# Autodesk Inventor assembly: GateLessMaterialAssembly
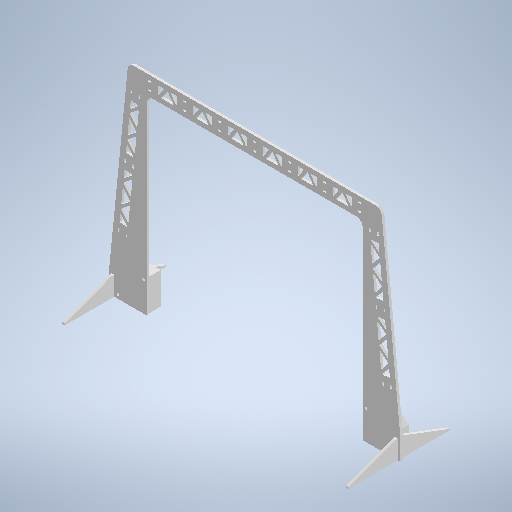
[picture p0: Inventor's stored thumbnail of the model, 512x512]
Saved by Autodesk Inventor 2025.1 (Build 291241000, 241)
## iProperties
Created: 2025-03-30
Part Number: GateLessMaterialAssembly
Document SubType Name: Assembly
Designer: 42060
Author: 42060
## Documents named in this file (4)
- C:\Users\42060\Desktop\School\Projects\RoboClash\LineFollower_Gate\GateLessMaterial\GateLessMaterialAssembly.iam
- C:\Users\42060\Desktop\School\Projects\RoboClash\LineFollower_Gate\GateLessMaterial\GateBrigeSideLessMaterial.ipt
- C:\Users\42060\Desktop\School\Projects\RoboClash\LineFollower_Gate\GateLessMaterial\LegLessMaterial.ipt
- C:\Users\42060\Desktop\School\Projects\RoboClash\LineFollower_Gate\GateLessMaterial\Sensor.ipt
## Components (5 placed, 3 different names)
1. GateBrigeSideLessMaterial:1 — Vložit:1, Vložit:2, Vložit:3, Vložit:4, Proti sobě:1, Proti sobě:2, Proti sobě:3, Proti sobě:4, Proti sobě:5, Proti sobě:6
2. LegLessMaterial:1 — Proti sobě:1, Proti sobě:2, Proti sobě:3
3. Sensor:1 — Vložit:1, Vložit:2
4. Sensor:2 — Vložit:3, Vložit:4
5. LegLessMaterial:2 — Proti sobě:4, Proti sobě:5, Proti sobě:6
## Relationships (10: Mate 6, Insert 4)
- Vložit:1 [Insert]: GateBrigeSideLessMaterial:1 ↔ Sensor:1
- Vložit:2 [Insert]: GateBrigeSideLessMaterial:1 ↔ Sensor:1
- Vložit:3 [Insert]: GateBrigeSideLessMaterial:1 ↔ Sensor:2
- Vložit:4 [Insert]: GateBrigeSideLessMaterial:1 ↔ Sensor:2
- Proti sobě:1 [Mate]: GateBrigeSideLessMaterial:1 ↔ LegLessMaterial:1
- Proti sobě:2 [Mate]: GateBrigeSideLessMaterial:1 ↔ LegLessMaterial:1
- Proti sobě:3 [Mate]: GateBrigeSideLessMaterial:1 ↔ LegLessMaterial:1
- Proti sobě:4 [Mate]: GateBrigeSideLessMaterial:1 ↔ LegLessMaterial:2
- Proti sobě:5 [Mate]: GateBrigeSideLessMaterial:1 ↔ LegLessMaterial:2
- Proti sobě:6 [Mate]: GateBrigeSideLessMaterial:1 ↔ LegLessMaterial:2
